# Autodesk Inventor assembly: 肩_1
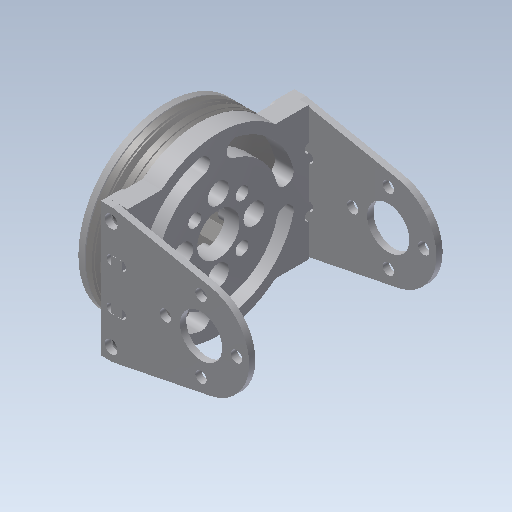
[picture p0: Inventor's stored thumbnail of the model, 512x512]
Saved by Autodesk Inventor 2020 (Build 240168000, 168)
## iProperties
Created: 2016-05-05
Part Number: 肩_1
Document SubType Name: Assembly
Designer: hiroaki
Mass: 31.2319 g
Surface Area: 187.261 cm^2
Volume: 14.2636 cm^3
Density: 2.18962 g/cm^3
Author: hiroaki
## Documents named in this file (7)
- C:\Users\Masato\Desktop\最新版\OpenPlatform_ver3_0\上半身\腕\肩_1.iam
- C:\Users\Masato\Desktop\最新版\OpenPlatform_ver3_0\上半身\腕\肩_メインフレーム_1_1.ipt
- C:\Users\Masato\Desktop\最新版\OpenPlatform_ver3_0\上半身\腕\肩_サブフレーム_1_1.ipt
- C:\Users\Masato\Desktop\最新版\OpenPlatform_ver3_0\Ready_Made\BA2542\core_BA2542.ipt
- C:\Users\Masato\Desktop\最新版\OpenPlatform_ver3_0\Ready_Made\BA2542\washer_BA2542.ipt
- C:\Users\Masato\Desktop\最新版\OpenPlatform_ver3_0\Ready_Made\MSU-306-03.ipt
- C:\Users\Masato\Desktop\最新版\OpenPlatform_ver3_0\上半身\腕\肩ピッチ_サブフレーム.ipt
## Components (11 placed, 6 different names)
1. 肩_メインフレーム_1_1:1 — 挿入:1, 挿入:2, 挿入:3, 挿入:4, 挿入:9, 挿入:16, 挿入:17, 挿入:18, 挿入:19
2. 肩_サブフレーム_1_1:1 — 挿入:3, 挿入:4
3. 肩_サブフレーム_1_1:2 — 挿入:1, 挿入:2
4. core_BA2542:1 — 挿入:10
5. washer_BA2542:1 — 挿入:9, 挿入:10
6. core_BA2542:2 — 挿入:20
7. MSU-306-03:1 — 挿入:16, 挿入:23
8. MSU-306-03:2 — 挿入:17, 挿入:24
9. MSU-306-03:3 — 挿入:18, 挿入:21
10. MSU-306-03:4 — 挿入:19, 挿入:22
11. 肩ピッチ_サブフレーム:1 — 挿入:20, 挿入:21, 挿入:22, 挿入:23, 挿入:24
## Relationships (15: Insert 15)
- 挿入:1 [Insert]: 肩_メインフレーム_1_1:1 ↔ 肩_サブフレーム_1_1:2
- 挿入:2 [Insert]: 肩_メインフレーム_1_1:1 ↔ 肩_サブフレーム_1_1:2
- 挿入:3 [Insert]: 肩_メインフレーム_1_1:1 ↔ 肩_サブフレーム_1_1:1
- 挿入:4 [Insert]: 肩_メインフレーム_1_1:1 ↔ 肩_サブフレーム_1_1:1
- 挿入:9 [Insert]: 肩_メインフレーム_1_1:1 ↔ washer_BA2542:1
- 挿入:10 [Insert]: core_BA2542:1 ↔ washer_BA2542:1
- 挿入:16 [Insert]: 肩_メインフレーム_1_1:1 ↔ MSU-306-03:1
- 挿入:17 [Insert]: 肩_メインフレーム_1_1:1 ↔ MSU-306-03:2
- 挿入:18 [Insert]: 肩_メインフレーム_1_1:1 ↔ MSU-306-03:3
- 挿入:19 [Insert]: 肩_メインフレーム_1_1:1 ↔ MSU-306-03:4
- 挿入:20 [Insert]: core_BA2542:2 ↔ 肩ピッチ_サブフレーム:1
- 挿入:21 [Insert]: MSU-306-03:3 ↔ 肩ピッチ_サブフレーム:1
- 挿入:22 [Insert]: MSU-306-03:4 ↔ 肩ピッチ_サブフレーム:1
- 挿入:23 [Insert]: MSU-306-03:1 ↔ 肩ピッチ_サブフレーム:1
- 挿入:24 [Insert]: MSU-306-03:2 ↔ 肩ピッチ_サブフレーム:1
